# Autodesk Inventor assembly: NewBasketAssemblie
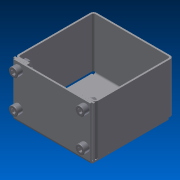
[picture p0: Inventor's stored thumbnail of the model, 180x180]
Saved by Autodesk Inventor 2013 (Build 170138000, 138)
## iProperties
Created: 2013-08-02
Part Number: NewBasketAssemblie
Document SubType Name: Assembly
Designer: nowireless
Author: nowireless
## Documents named in this file (5)
- J:\FRC_Projects\Cad\Inventor_Projects\Shooter_No_Welding\Thrower\NewBasketAssemblie.iam
- J:\FRC_Projects\Cad\Inventor_Projects\Shooter_No_Welding\Thrower\NewBasket.ipt
- J:\FRC_Projects\Cad\Inventor_Projects\Shooter_No_Welding\Thrower\SpacerBasket.ipt
- J:\FRC_Projects\Cad\Inventor_Projects\Shooter_No_Welding\contentCenter\en-US\ANSI B 18.2.4.1 M(1)\ANSI B 18.2.4.1 M - M5 x 0.8Style 1.ipt
- J:\FRC_Projects\Cad\Inventor_Projects\Shooter_No_Welding\contentCenter\en-US\ANSI B18.3.1M(1)\ANSI B18.3.1M - M5x0.8 x 10(2).ipt
## Components (11 placed, 4 different names)
1. NewBasket:1 — Mate:1, Mate:2, Mate:3, Mate:4, Mate:5, Mate:6, Mate:7, Mate:8, Mate:9, Mate:10, Mate:11, Mate:12, Mate:13, Mate:14, Mate:16, Mate:18, Mate:20, Mate:22
2. SpacerBasket:1 — Mate:1, Mate:2, Mate:3
3. SpacerBasket:2 — Mate:4, Mate:5, Mate:6
4. Broached Socket Head Cap Screw - Metric M5x0.8 x 10:3 — Mate:10, Mate:13, Mate:17
5. Broached Socket Head Cap Screw - Metric M5x0.8 x 10:2 — Mate:9, Mate:14, Mate:21
6. Broached Socket Head Cap Screw - Metric M5x0.8 x 10:1 — Mate:7, Mate:8, Mate:15
7. Broached Socket Head Cap Screw - Metric M5x0.8 x 10:4 — Mate:11, Mate:12, Mate:19
8. Hex Nut Metric M5 x 0.8:1 — Mate:17, Mate:18
9. Hex Nut Metric M5 x 0.8:2 — Mate:15, Mate:16
10. Hex Nut Metric M5 x 0.8:3 — Mate:19, Mate:20
11. Hex Nut Metric M5 x 0.8:4 — Mate:21, Mate:22
## Relationships (22: Mate 22)
- Mate:1: NewBasket:1 ↔ SpacerBasket:1
- Mate:2: NewBasket:1 ↔ SpacerBasket:1
- Mate:3: NewBasket:1 ↔ SpacerBasket:1
- Mate:4: NewBasket:1 ↔ SpacerBasket:2
- Mate:5: NewBasket:1 ↔ SpacerBasket:2
- Mate:6: NewBasket:1 ↔ SpacerBasket:2
- Mate:7: NewBasket:1 ↔ Broached Socket Head Cap Screw - Metric M5x0.8 x 10:1
- Mate:8: NewBasket:1 ↔ Broached Socket Head Cap Screw - Metric M5x0.8 x 10:1
- Mate:9: NewBasket:1 ↔ Broached Socket Head Cap Screw - Metric M5x0.8 x 10:2
- Mate:10: NewBasket:1 ↔ Broached Socket Head Cap Screw - Metric M5x0.8 x 10:3
- Mate:11: NewBasket:1 ↔ Broached Socket Head Cap Screw - Metric M5x0.8 x 10:4
- Mate:12: NewBasket:1 ↔ Broached Socket Head Cap Screw - Metric M5x0.8 x 10:4
- Mate:13: NewBasket:1 ↔ Broached Socket Head Cap Screw - Metric M5x0.8 x 10:3
- Mate:14: NewBasket:1 ↔ Broached Socket Head Cap Screw - Metric M5x0.8 x 10:2
- Mate:15: Broached Socket Head Cap Screw - Metric M5x0.8 x 10:1 ↔ Hex Nut Metric M5 x 0.8:2
- Mate:16: NewBasket:1 ↔ Hex Nut Metric M5 x 0.8:2
- Mate:17: Broached Socket Head Cap Screw - Metric M5x0.8 x 10:3 ↔ Hex Nut Metric M5 x 0.8:1
- Mate:18: NewBasket:1 ↔ Hex Nut Metric M5 x 0.8:1
- Mate:19: Broached Socket Head Cap Screw - Metric M5x0.8 x 10:4 ↔ Hex Nut Metric M5 x 0.8:3
- Mate:20: NewBasket:1 ↔ Hex Nut Metric M5 x 0.8:3
- Mate:21: Broached Socket Head Cap Screw - Metric M5x0.8 x 10:2 ↔ Hex Nut Metric M5 x 0.8:4
- Mate:22: NewBasket:1 ↔ Hex Nut Metric M5 x 0.8:4
